# Autodesk Inventor assembly: Left_Arm
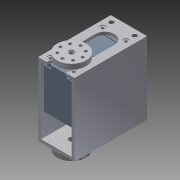
[picture p0: Inventor's stored thumbnail of the model, 180x180]
Saved by Autodesk Inventor 2013 (Build 170138000, 138)
## iProperties
Created: 2014-05-07
Part Number: Left_Arm
Document SubType Name: Assembly
Designer: andou
Author: andou
## Documents named in this file (6)
- C:\Users\andou\Documents\Inventor\RoboticsProject\project_4\Robot\Arm\Left_Arm.iam
- C:\Users\andou\Documents\Inventor\RoboticsProject\project_4\Robot\All Common\Serial_Case.ipt
- C:\Users\andou\Documents\Inventor\RoboticsProject\project_4\Robot\Arm\KRS-2542HV.ipt
- C:\Users\andou\Documents\Inventor\RoboticsProject\project_4\Robot\Free_Horn\Free_Horn.iam
- C:\Users\andou\Documents\Inventor\RoboticsProject\project_4\Robot\All Common\Low_Height_Horn.ipt
- C:\Users\andou\Documents\Inventor\RoboticsProject\project_4\Robot\Arm\Horn_Spacer.ipt
## Components (5 placed, 5 different names)
1. Serial_Case:1 — 挿入:1, 挿入:9, 挿入:10
2. Free_Horn:1 [sub-assembly] — 挿入:1
3. KRS-2542HV:1 — 挿入:8, 挿入:9, 挿入:10
4. Low_Height_Horn:1 — 挿入:8, 挿入:11, 挿入:12
5. Horn_Spacer:1 — 挿入:11, 挿入:12
## Relationships (6: Insert 6)
- 挿入:1 [Insert]: Serial_Case:1 ↔ Free_Horn:1
- 挿入:8 [Insert]: KRS-2542HV:1 ↔ Low_Height_Horn:1
- 挿入:9 [Insert]: Serial_Case:1 ↔ KRS-2542HV:1
- 挿入:10 [Insert]: Serial_Case:1 ↔ KRS-2542HV:1
- 挿入:11 [Insert]: Low_Height_Horn:1 ↔ Horn_Spacer:1
- 挿入:12 [Insert]: Low_Height_Horn:1 ↔ Horn_Spacer:1
